# Autodesk Inventor assembly: Assembly9
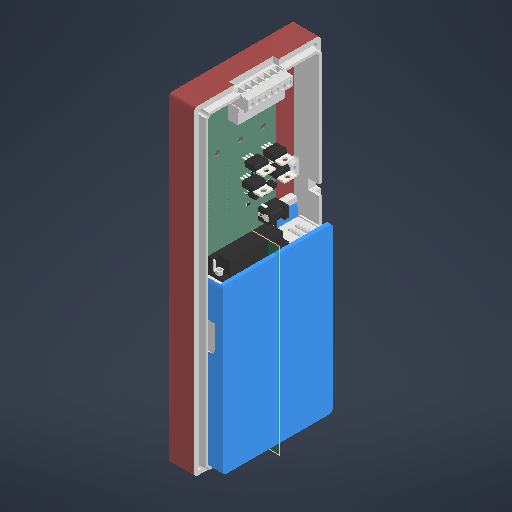
[picture p0: Inventor's stored thumbnail of the model, 512x512]
Saved by Autodesk Inventor 2027 (Build 310192000, 192)
## iProperties
Created: 2026-05-22
Part Number: Assembly9
Document SubType Name: Assembly
Designer: giese
Author: giese
## Documents named in this file (5)
- C:\Users\giese\OneDrive\Documents\GitHub\Biphasic-data-acquisition-system\DAQ_design\Assisi\v0.2.1\CAD\Assembly9.iam
- C:\Users\giese\OneDrive\Documents\GitHub\Biphasic-data-acquisition-system\DAQ_design\Assisi\v0.2.1\CAD\cDAQ_Bottom_Box3.ipt
- C:\Users\giese\OneDrive\Documents\GitHub\Biphasic-data-acquisition-system\DAQ_design\Assisi\v0.2.1\CAD\cDAQ_Chassis_LowPolyPlaceholder.ipt
- C:\Users\giese\OneDrive\Documents\GitHub\Biphasic-data-acquisition-system\DAQ_design\Assisi\v0.2.1\EDA\assisi_v0.2.1_NEW\assisi_v0.2.1_NEW.ipt
- C:\Users\giese\OneDrive\Documents\GitHub\Biphasic-data-acquisition-system\DAQ_design\Assisi\v0.2.1\CAD\cdaq\cdaq.ipt
## Components (4 placed, 4 different names)
1. cDAQ_Bottom_Box3:1 — Mate:19, Mate:21, Mate:22, Mate:27
2. cDAQ_Chassis_LowPolyPlaceholder:1 — Mate:19, Mate:21, Mate:22, Mate:23, Mate:24, Mate:25
3. cdaq:1 — Mate:23, Mate:24, Mate:25, Mate:26, Mate:28
4. assisi_v0.2.1_NEW:1 — Mate:26, Mate:27, Mate:28
## Relationships (9: Mate 9)
- Mate:19: cDAQ_Bottom_Box3:1 ↔ cDAQ_Chassis_LowPolyPlaceholder:1
- Mate:21: cDAQ_Bottom_Box3:1 ↔ cDAQ_Chassis_LowPolyPlaceholder:1
- Mate:22: cDAQ_Bottom_Box3:1 ↔ cDAQ_Chassis_LowPolyPlaceholder:1
- Mate:23: cDAQ_Chassis_LowPolyPlaceholder:1 ↔ cdaq:1
- Mate:24: cDAQ_Chassis_LowPolyPlaceholder:1 ↔ cdaq:1
- Mate:25: cDAQ_Chassis_LowPolyPlaceholder:1 ↔ cdaq:1
- Mate:26: cdaq:1 ↔ assisi_v0.2.1_NEW:1
- Mate:27: cDAQ_Bottom_Box3:1 ↔ assisi_v0.2.1_NEW:1
- Mate:28: cdaq:1 ↔ assisi_v0.2.1_NEW:1
